# Autodesk Inventor assembly: ASY Disk Micro filter
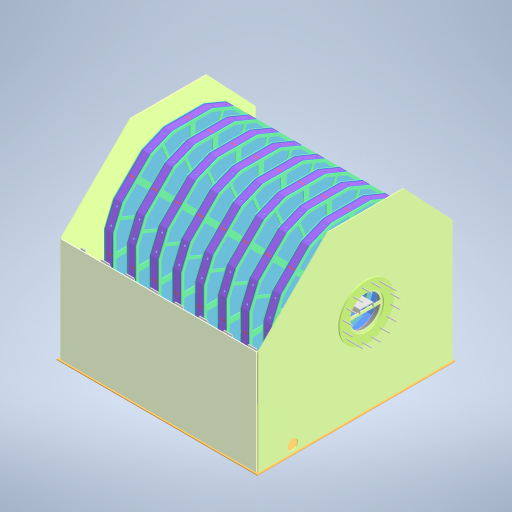
[picture p0: Inventor's stored thumbnail of the model, 512x512]
Saved by Autodesk Inventor 2024.2 (Build 282272000, 272)
## iProperties
Created: 2023-08-31
Part Number: ASY Disk Micro filter
Document SubType Name: Assembly
Designer: admin
Stock Number: Дисковый_Фильтр
Author: admin
## Documents named in this file (27)
- C:\Users\user\YandexDisk\домашниий пк\Inventor\DMF-Disk-Micro-Filter\ASY 000 ДМФ Disk Micro filter.iam
- C:\Users\user\YandexDisk\домашниий пк\Inventor\DMF-Disk-Micro-Filter\Left wall.ipt
- C:\Users\user\YandexDisk\домашниий пк\Inventor\DMF-Disk-Micro-Filter\Wall right.ipt
- C:\Users\user\YandexDisk\домашниий пк\Inventor\DMF-Disk-Micro-Filter\DF1.03 Wall bottom.ipt
- C:\Users\user\YandexDisk\домашниий пк\Inventor\DMF-Disk-Micro-Filter\DF1.04 Wall face.ipt
- C:\Users\user\YandexDisk\домашниий пк\Inventor\DMF-Disk-Micro-Filter\ыASY xDF frame.iam
- C:\Users\user\YandexDisk\домашниий пк\Inventor\DMF-Disk-Micro-Filter\ДМФ 021 кольцо прижимное нос.ipt
- C:\Users\user\YandexDisk\домашниий пк\Inventor\DMF-Disk-Micro-Filter\ДМФ 000 размеры.ipt
- C:\Users\user\YandexDisk\домашниий пк\Inventor\DMF-Disk-Micro-Filter\ASY ДМФ 030 кольцо со шпильками корма.iam
- C:\Users\user\YandexDisk\домашниий пк\Inventor\DMF-Disk-Micro-Filter\ДМФ 032 крышка Нос.ipt
- C:\Users\user\YandexDisk\домашниий пк\Inventor\DMF-Disk-Micro-Filter\ASY ДМФ 0100 Барабан.iam
- C:\Users\user\YandexDisk\домашниий пк\Inventor\DMF-Disk-Micro-Filter\ДМФ 091 Постель НОС.ipt
- C:\Users\user\YandexDisk\домашниий пк\Inventor\DMF-Disk-Micro-Filter\ASY ДМФ 040 кольцо под шпильки КОРМА.iam
- C:\Users\user\YandexDisk\домашниий пк\Inventor\DMF-Disk-Micro-Filter\ДМФ 022 кольцо прижимное корма.ipt
- C:\Users\user\YandexDisk\домашниий пк\Inventor\DMF-Disk-Micro-Filter\ДМФ 093 Постель КОРМА.ipt
- C:\Users\user\YandexDisk\домашниий пк\Inventor\DMF-Disk-Micro-Filter\ДМФ 092 Коромысло КОРМА.ipt
- C:\Users\user\YandexDisk\домашниий пк\Inventor\DMF-Disk-Micro-Filter\ДМФ 055 труба илоотвода.ipt
- C:\Users\user\YandexDisk\домашниий пк\Inventor\DMF-Disk-Micro-Filter\ДМФ 033 держатель лотка.ipt
- C:\Users\user\YandexDisk\домашниий пк\Inventor\DMF-Disk-Micro-Filter\ASY ДМФ лоток 050 илоотвод.iam
- C:\Users\user\YandexDisk\домашниий пк\Inventor\DMF-Disk-Micro-Filter\ДМФ 092 Коромысло НОС.ipt
- C:\Users\user\YandexDisk\домашниий пк\Inventor\DMF-Disk-Micro-Filter\ДМФ 011 Стенка Корма ЛЕВ.ipt
- C:\Users\user\YandexDisk\домашниий пк\Inventor\DMF-Disk-Micro-Filter\ДМФ 012 Стенка Корма ПРАВ.ipt
- C:\Users\user\YandexDisk\домашниий пк\Inventor\DMF-Disk-Micro-Filter\ДМФ 014 Стенка Нос ЛЕВ.ipt
- C:\Users\user\YandexDisk\домашниий пк\Inventor\DMF-Disk-Micro-Filter\ДМФ 015 Стенка Нос ПРАВ.ipt
- C:\Users\user\YandexDisk\домашниий пк\Inventor\DMF-Disk-Micro-Filter\ДМФ 066 Гребенка.ipt
- C:\Users\user\YandexDisk\домашниий пк\Inventor\DMF-Disk-Micro-Filter\ДМФ 025 кольцо прижимное корма наружное.ipt
- C:\Users\user\YandexDisk\домашниий пк\Inventor\DMF-Disk-Micro-Filter\ASY ДМФ 070 кольцо под шпильки КОРМА наружное.iam
## Components (26 placed, 26 different names)
1. ДМФ 000 размеры:1
2. Left wall:1 — Flush:3, Flush:4, Mate:1, Flush:6, Flush:7, Flush:9, Mate:4, Flush:16, Rotational:12, Rigid:9, Rigid:12
3. Wall right:1 — Flush:3, Mate:2, Flush:8, Mate:22, Rigid:14
4. DF1.03 Wall bottom:1 — Mate:1, Mate:2, Flush:6, Flush:7, Flush:8, Mate:3, Flush:11, Mate:5, Mate:24
5. DF1.04 Wall face:1 — Flush:9, Mate:3, Mate:4, Flush:10, Angle:1
6. ASY DF frame:1 [sub-assembly] — Flush:15, Flush:13, Flush:14, Mate:5
7. ДМФ 021 кольцо прижимное нос:1 — Rotational:12, Mate:13, Rotational:14
8. ASY ДМФ 030 кольцо со шпильками корма:1 [sub-assembly] — Flush:16, Rigid:9
9. ДМФ 032 крышка Нос:1 — Mate:16, Rigid:8, Rigid:12
10. ASY ДМФ 0100 Барабан:1 [sub-assembly] — Rotational:15
11. ДМФ 091 Постель НОС:2 — Flush:17, Rotational:14, Rigid:10, Rotational:15
12. ASY ДМФ 101 кольцо со шпильками корма:1 [sub-assembly] — Mate:14, Rigid:13
13. ДМФ 022 кольцо прижимное корма:1 — Flush:18, Rigid:11, Rigid:13
14. ДМФ 093 Постель КОРМА:1 — Mate:15, Rigid:3, Rigid:11
15. Постель 204 корма:1 — Rigid:3
16. ДМФ 055 труба илоотвода:1 — Rigid:8, Tangent:1
17. ДМФ 033 держатель лотка:1 — Mate:16, Mate:17, Tangent:1, Mate:23
18. ASY ДМФ лоток 050 илоотвод:1 [sub-assembly] — Mate:22, Mate:23
19. ДМФ 092 Коромысло НОС:1 — Rigid:10
20. ДМФ 011 Стенка Корма ЛЕВ:1
21. ДМФ 012 Стенка Корма ПРАВ:1
22. ДМФ 014 Стенка Нос ЛЕВ:1
23. ДМФ 015 Стенка Нос ПРАВ:1
24. ДМФ 066 Гребенка:1 — Flush:22, Angle:1, Mate:24
25. ДМФ 025 кольцо прижимное корма наружное:1 — Rigid:14, Rigid:15
26. ASY ДМФ 070 кольцо под шпильки КОРМА наружное:1 [sub-assembly] — Rigid:15
## Relationships (44: Flush 16, Mate 14, WeldJoint 9, RevoluteJoint 3, Tangent 1, Angle 1)
- Flush:3: Left wall:1 ↔ Wall right:1
- Flush:4: Left wall:1
- Mate:1: Left wall:1 ↔ DF1.03 Wall bottom:1
- Mate:2: Wall right:1 ↔ DF1.03 Wall bottom:1
- Flush:6 (15 mm): Left wall:1 ↔ DF1.03 Wall bottom:1
- Flush:7 (25 mm): Left wall:1 ↔ DF1.03 Wall bottom:1
- Flush:8 (15 mm): Wall right:1 ↔ DF1.03 Wall bottom:1
- Flush:9: Left wall:1 ↔ DF1.04 Wall face:1
- Mate:3: DF1.03 Wall bottom:1 ↔ DF1.04 Wall face:1
- Mate:4: Left wall:1 ↔ DF1.04 Wall face:1
- Flush:10: DF1.04 Wall face:1
- Flush:11: DF1.03 Wall bottom:1
- [Flush]: ASY DF frame:1
- Flush:15: ASY DF frame:1
- Flush:13: ASY DF frame:1
- Flush:14: ASY DF frame:1
- Mate:5: DF1.03 Wall bottom:1 ↔ ASY DF frame:1
- Flush:16: Left wall:1 ↔ ASY ДМФ 030 кольцо со шпильками корма:1
- Rotational:12 [RevoluteJoint]: Left wall:1 ↔ ДМФ 021 кольцо прижимное нос:1
- Mate:13: ДМФ 021 кольцо прижимное нос:1
- Flush:17: ДМФ 091 Постель НОС:2
- Mate:14: ASY ДМФ 101 кольцо со шпильками корма:1
- Flush:18: ДМФ 022 кольцо прижимное корма:1
- Mate:15: ДМФ 093 Постель КОРМА:1
- Rigid:3 [WeldJoint]: ДМФ 093 Постель КОРМА:1 ↔ Постель 204 корма:1
- [Mate]: ASY ДМФ лоток 050 илоотвод:1
- Mate:16: ДМФ 032 крышка Нос:1 ↔ ДМФ 033 держатель лотка:1
- Mate:17: ДМФ 033 держатель лотка:1
- Rigid:8 [WeldJoint]: ДМФ 032 крышка Нос:1 ↔ ДМФ 055 труба илоотвода:1
- Rigid:9 [WeldJoint]: Left wall:1 ↔ ASY ДМФ 030 кольцо со шпильками корма:1
- Tangent:1: ДМФ 055 труба илоотвода:1 ↔ ДМФ 033 держатель лотка:1
- Mate:22: Wall right:1 ↔ ASY ДМФ лоток 050 илоотвод:1
- Mate:23: ДМФ 033 держатель лотка:1 ↔ ASY ДМФ лоток 050 илоотвод:1
- Rotational:14 [RevoluteJoint]: ДМФ 021 кольцо прижимное нос:1 ↔ ДМФ 091 Постель НОС:2
- Rigid:10 [WeldJoint]: ДМФ 091 Постель НОС:2 ↔ ДМФ 092 Коромысло НОС:1
- Rotational:15 [RevoluteJoint]: ASY ДМФ 0100 Барабан:1 ↔ ДМФ 091 Постель НОС:2
- Rigid:11 [WeldJoint]: ДМФ 022 кольцо прижимное корма:1 ↔ ДМФ 093 Постель КОРМА:1
- Rigid:12 [WeldJoint]: Left wall:1 ↔ ДМФ 032 крышка Нос:1
- Flush:22: ДМФ 066 Гребенка:1
- Angle:1 (180 deg): DF1.04 Wall face:1 ↔ ДМФ 066 Гребенка:1
- Mate:24: DF1.03 Wall bottom:1 ↔ ДМФ 066 Гребенка:1
- Rigid:13 [WeldJoint]: ASY ДМФ 101 кольцо со шпильками корма:1 ↔ ДМФ 022 кольцо прижимное корма:1
- Rigid:14 [WeldJoint]: Wall right:1 ↔ ДМФ 025 кольцо прижимное корма наружное:1
- Rigid:15 [WeldJoint]: ДМФ 025 кольцо прижимное корма наружное:1 ↔ ASY ДМФ 070 кольцо под шпильки КОРМА наружное:1
